# Autodesk Inventor assembly: ISO63
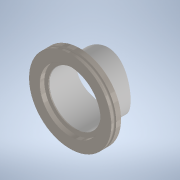
[picture p0: Inventor's stored thumbnail of the model, 180x180]
Saved by Autodesk Inventor 2021 (Build 250183000, 183)
## iProperties
Created: 2024-04-12
Part Number: ISO63
Document SubType Name: Assembly
Designer: Sebastián
Author: Sebastián
## Documents named in this file (3)
- C:\Users\Sebastián\Documents\Inventor\PLD SAP\ISO63.iam
- C:\Users\Sebastián\Documents\Inventor\PLD SAP\ISO63_flange.ipt
- C:\Users\Sebastián\Documents\Inventor\PLD_Chamber\Hositrad_ISO-K63-64.ipt
## Components (2 placed, 2 different names)
1. ISO63_flange:1 — Rigid:1
2. Hositrad_ISO-K63-64:1 — Rigid:1
## Relationships (1: WeldJoint 1)
- Rigid:1 [WeldJoint]: ISO63_flange:1 ↔ Hositrad_ISO-K63-64:1
